# Autodesk Inventor assembly: Motorhalterung_komplett
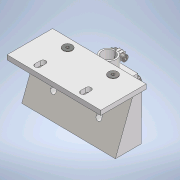
[picture p0: Inventor's stored thumbnail of the model, 180x180]
Saved by Autodesk Inventor 2020.1 (Build 241239000, 239)
## iProperties
Created: 2020-08-19
Part Number: Motorhalterung_komplett
Document SubType Name: Assembly
Designer: s5chfeis
Author: s5chfeis
## Documents named in this file (9)
- Z:\Masterarbeit\CAD\CAD\Motorhalterung_komplett.iam
- Z:\Masterarbeit\CAD\CAD\Motorhalterung_BT1.ipt
- Z:\Masterarbeit\CAD\CAD\Motorhalterung_BT2.1.ipt
- d:\Users\s5chfeis\Documents\Inventor\Content Center Files\R2020\de-DE\BS 4168(8)\BS 4168 - M10 x 30(7).ipt
- Z:\Masterarbeit\CAD\CAD\Hülse.ipt
- Z:\Masterarbeit\CAD\CAD\Motorhalterung_BT3.ipt
- d:\Users\s5chfeis\Documents\Inventor\Content Center Files\R2020\de-DE\AS 1420\AS 1420 - 1973 - M10 x 45.ipt
- d:\Users\s5chfeis\Documents\Inventor\Content Center Files\R2020\de-DE\AS 1420\AS 1420 - 1973 - M8 x 25.ipt
- d:\Users\s5chfeis\Documents\Inventor\Content Center Files\R2020\de-DE\AS 1112 (2)\AS 1112 - M8  Typ 8.ipt
## Components (12 placed, 8 different names)
1. Motorhalterung_BT1:1 — Passend:1, Passend:2, Passend:3, Passend:6
2. Motorhalterung_BT2.1:1 — Passend:1, Passend:4, Passend:5, Passend:6, Passend:7, Passend:8
3. BS 4168 : Teil 8 Senkkopf- und Halbrundschrauben mit Innensechskant - metrische Ausführung - Metrisch M10 x 30:1 — Passend:2
4. BS 4168 : Teil 8 Senkkopf- und Halbrundschrauben mit Innensechskant - metrische Ausführung - Metrisch M10 x 30:2 — Passend:3
5. Hülse:1 — Passend:4, Passend:5, Einfügen:3, Einfügen:4, Passend:10, Passend:12
6. Motorhalterung_BT3:1 — Passend:7, Passend:8, Einfügen:1, Einfügen:2
7. AS 1420 - Metrisch M10 x 45:1 — Einfügen:1
8. AS 1420 - Metrisch M10 x 45:2 — Einfügen:2
9. AS 1420 - Metrisch M8 x 25:1 — Einfügen:3, Passend:9
10. AS 1420 - Metrisch M8 x 25:2 — Einfügen:4, Passend:11
11. AS 1112 (2) - Metrisch M8  Typ 8:1 — Passend:9, Passend:10
12. AS 1112 (2) - Metrisch M8  Typ 8:2 — Passend:11, Passend:12
## Relationships (16: Mate 12, Insert 4)
- Passend:1 [Mate]: Motorhalterung_BT1:1 ↔ Motorhalterung_BT2.1:1
- Passend:2 [Mate]: Motorhalterung_BT1:1 ↔ BS 4168 : Teil 8 Senkkopf- und Halbrundschrauben mit Innensechskant - metrische Ausführung - Metrisch M10 x 30:1
- Passend:3 [Mate]: Motorhalterung_BT1:1 ↔ BS 4168 : Teil 8 Senkkopf- und Halbrundschrauben mit Innensechskant - metrische Ausführung - Metrisch M10 x 30:2
- Passend:4 [Mate]: Motorhalterung_BT2.1:1 ↔ Hülse:1
- Passend:5 [Mate]: Motorhalterung_BT2.1:1 ↔ Hülse:1
- Passend:6 [Mate]: Motorhalterung_BT1:1 ↔ Motorhalterung_BT2.1:1
- Passend:7 [Mate]: Motorhalterung_BT2.1:1 ↔ Motorhalterung_BT3:1
- Passend:8 [Mate]: Motorhalterung_BT2.1:1 ↔ Motorhalterung_BT3:1
- Einfügen:1 [Insert]: Motorhalterung_BT3:1 ↔ AS 1420 - Metrisch M10 x 45:1
- Einfügen:2 [Insert]: Motorhalterung_BT3:1 ↔ AS 1420 - Metrisch M10 x 45:2
- Einfügen:3 [Insert]: Hülse:1 ↔ AS 1420 - Metrisch M8 x 25:1
- Einfügen:4 [Insert]: Hülse:1 ↔ AS 1420 - Metrisch M8 x 25:2
- Passend:9 [Mate]: AS 1420 - Metrisch M8 x 25:1 ↔ AS 1112 (2) - Metrisch M8  Typ 8:1
- Passend:10 [Mate]: Hülse:1 ↔ AS 1112 (2) - Metrisch M8  Typ 8:1
- Passend:11 [Mate]: AS 1420 - Metrisch M8 x 25:2 ↔ AS 1112 (2) - Metrisch M8  Typ 8:2
- Passend:12 [Mate]: Hülse:1 ↔ AS 1112 (2) - Metrisch M8  Typ 8:2
